# Autodesk Inventor assembly: holder
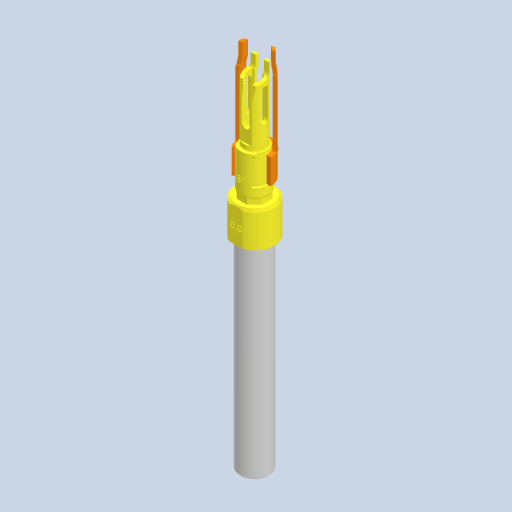
[picture p0: Inventor's stored thumbnail of the model, 512x512]
Saved by Autodesk Inventor 2024 (Build 280153000, 153)
## iProperties
Created: 2023-06-15
Part Number: holder
Document SubType Name: Assembly
Designer: dsdan
Author: dsdan
## Documents named in this file (4)
- E:\OneDrive - Imperial College London\DragonVision_DanielKo\Instrumentation\Ephys_rig_2021\holder.iam
- E:\OneDrive - Imperial College London\DragonVision_DanielKo\Instrumentation\Ephys_rig_2021\Holder\body_adjustable_parametric_thorlabs.ipt
- E:\OneDrive - Imperial College London\DragonVision_DanielKo\Instrumentation\Ephys_rig_2021\Holder\head_adjustable_v5.ipt
- E:\OneDrive - Imperial College London\DragonVision_DanielKo\Instrumentation\Ephys_rig_2021\Imported Components\TR100_M-Solidworks.ipt
## Components (3 placed, 3 different names)
1. body_adjustable_parametric_thorlabs:1 — Mate:1, Mate:2, Mate:5, Mate:6
2. head_adjustable_v5:1 — Mate:1, Mate:2
3. TR100_M-Solidworks:1 — Mate:5, Mate:6
## Relationships (4: Mate 4)
- Mate:1: body_adjustable_parametric_thorlabs:1 ↔ head_adjustable_v5:1
- Mate:2: body_adjustable_parametric_thorlabs:1 ↔ head_adjustable_v5:1
- Mate:5: body_adjustable_parametric_thorlabs:1 ↔ TR100_M-Solidworks:1
- Mate:6: body_adjustable_parametric_thorlabs:1 ↔ TR100_M-Solidworks:1
